# Autodesk Inventor assembly: 9P Sprocket
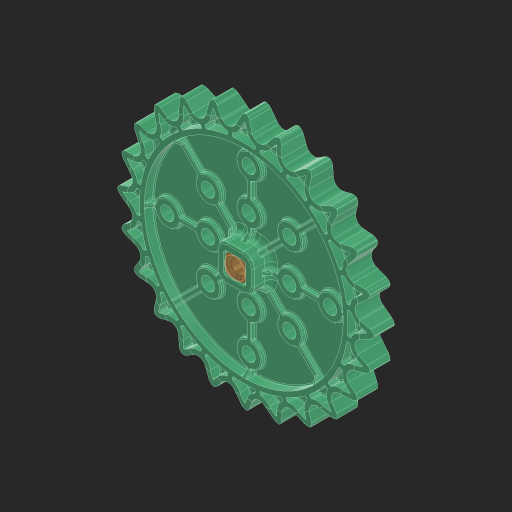
[picture p0: Inventor's stored thumbnail of the model, 512x512]
Saved by Autodesk Inventor 2023 (Build 270158000, 158)
## iProperties
Created: 2022-08-02
Part Number: 9P Sprocket
Document SubType Name: Assembly
Designer: ylu12
Author: ylu12
## Documents named in this file (4)
- C:\Users\ylu12\Documents\GitHub\VEX-CAD-Inventor\Motion\Sprockets\9P Sprocket\9P 24T Sprocket, Circle.iam
- C:\Users\ylu12\Documents\GitHub\VEX-CAD-Inventor\Motion\HS Shaft Adapter Circle.ipt
- C:\Users\ylu12\Documents\GitHub\VEX-CAD-Inventor\Motion\Sprockets\Reference Files\9P 24T Sprocket, No Insert.ipt
- C:\Users\ylu12\Documents\GitHub\VEX-CAD-Inventor\Motion\Sprockets\9P Sprocket.iam
## Components (2 placed, 2 different names)
1. Circle — Mate:1, Mate:2, Flush:1
2. 24T — Flush:6, Mate:11, Mate:12
## Relationships (6: Mate 4, Flush 2)
- Mate:1: Circle
- Mate:2: Circle
- Flush:1 (6.35 mm): Circle
- Flush:6: 24T
- Mate:11: 24T
- Mate:12: 24T
